# Autodesk Inventor assembly: Chain
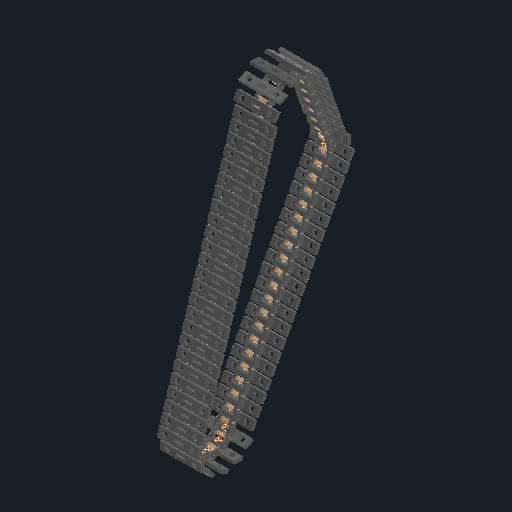
[picture p0: Inventor's stored thumbnail of the model, 512x512]
Saved by Autodesk Inventor 2025 (Build 290162000, 162)
## iProperties
Created: 2024-10-20
Part Number: Chain
Document SubType Name: Assembly
Designer: Averey Ku
Author: Averey Ku
## Documents named in this file (3)
- D:\VEX\High Stakes\CAD\V2\Hook\Chain.iam
- D:\VEX\High Stakes\CAD\V2\Hook\Chain Path.ipt
- D:\VEX\High Stakes\CAD\ROBOPROS-CAD-Inventor\Motion\Chain 9P\Chain Attachment Link.ipt
## Components (64 placed, 2 different names)
1. Chain Path:1
2. Chain Attachment Link:1
3. Chain Attachment Link:2
4. Chain Attachment Link:3
5. Chain Attachment Link:4
6. Chain Attachment Link:5
7. Chain Attachment Link:6
8. Chain Attachment Link:7
9. Chain Attachment Link:8
10. Chain Attachment Link:9
11. Chain Attachment Link:10
12. Chain Attachment Link:11
13. Chain Attachment Link:12
14. Chain Attachment Link:13
15. Chain Attachment Link:14
16. Chain Attachment Link:15
17. Chain Attachment Link:16
18. Chain Attachment Link:17
19. Chain Attachment Link:18
20. Chain Attachment Link:19
21. Chain Attachment Link:20
22. Chain Attachment Link:21
23. Chain Attachment Link:22
24. Chain Attachment Link:23
25. Chain Attachment Link:24
26. Chain Attachment Link:25
27. Chain Attachment Link:26
28. Chain Attachment Link:27
29. Chain Attachment Link:28
30. Chain Attachment Link:29
31. Chain Attachment Link:30
32. Chain Attachment Link:31
33. Chain Attachment Link:32
34. Chain Attachment Link:33
35. Chain Attachment Link:34
36. Chain Attachment Link:35
37. Chain Attachment Link:36
38. Chain Attachment Link:37
39. Chain Attachment Link:38
40. Chain Attachment Link:39
41. Chain Attachment Link:40
42. Chain Attachment Link:41
43. Chain Attachment Link:42
44. Chain Attachment Link:43
45. Chain Attachment Link:44
46. Chain Attachment Link:45
47. Chain Attachment Link:46
48. Chain Attachment Link:47
49. Chain Attachment Link:48
50. Chain Attachment Link:49
51. Chain Attachment Link:50
52. Chain Attachment Link:51
53. Chain Attachment Link:52
54. Chain Attachment Link:53
55. Chain Attachment Link:54
56. Chain Attachment Link:55
57. Chain Attachment Link:56
58. Chain Attachment Link:57
59. Chain Attachment Link:58
60. Chain Attachment Link:59
61. Chain Attachment Link:60
62. Chain Attachment Link:61
63. Chain Attachment Link:62
64. Chain Attachment Link:63
## Component patterns: Links (63 elements)
